# Autodesk Inventor assembly: HUDSON-1-49
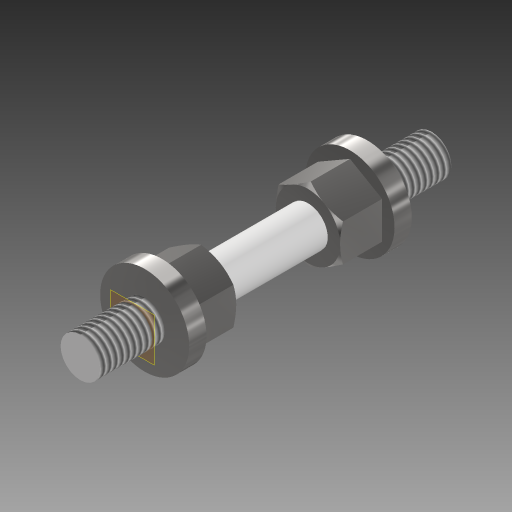
[picture p0: Inventor's stored thumbnail of the model, 512x512]
Saved by Autodesk Inventor 2024.2 (Build 282272000, 272)
## iProperties
Created: 2024-10-10
Part Number: HUDSON-1-49
Document SubType Name: Assembly
Designer: Precisión-05
Author: Precisión-05
## Documents named in this file (3)
- C:\Users\Precisión-05\Desktop\LOCOMOTORA CABALLERO\HUDSON-1-49.iam
- C:\Users\Precisión-05\Desktop\LOCOMOTORA CABALLERO\HUDSON-1-49A.ipt
- C:\Users\Precisión-05\Documents\Inventor\Content Center Files\R2024\en-US\DIN 6331\DIN 6331 - M 8.ipt
## Components (3 placed, 2 different names)
1. HUDSON-1-49A:1 — Rigid:1, Rigid:2
2. DIN 6331 M 8:1 — Rigid:1
3. DIN 6331 M 8:2 — Rigid:2
## Relationships (2: WeldJoint 2)
- Rigid:1 [WeldJoint] (-25 mm): HUDSON-1-49A:1 ↔ DIN 6331 M 8:1
- Rigid:2 [WeldJoint] (-25 mm): HUDSON-1-49A:1 ↔ DIN 6331 M 8:2
